# Autodesk Inventor assembly: XL,XC-330
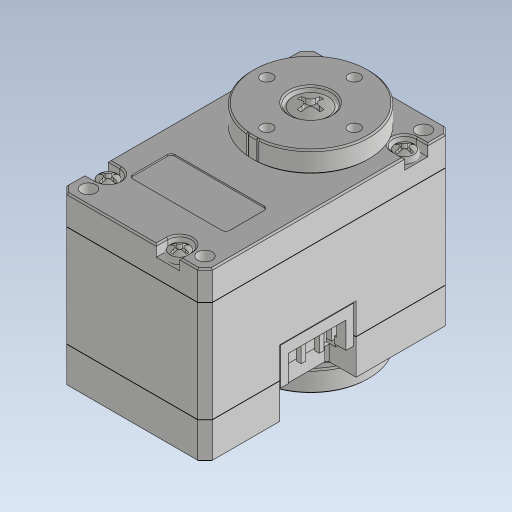
[picture p0: Inventor's stored thumbnail of the model, 512x512]
Saved by Autodesk Inventor 2023 (Build 270158000, 158)
## iProperties
Created: 2020-07-27
Part Number: XL,XC-330
Document SubType Name: Assembly
Designer: michi
Sending System: CREO PARAMETRIC BY PTC INC, 2019224
Preprocessor: CREO PARAMETRIC BY PTC INC, 2019224
Title: DC15_A01_DUMMY_ASSY_IDLE_ASM
Author: yunever
Revision Number: 9LAST_VERSION
## Documents named in this file (11)
- C:\Users\michi\OneDrive - Kyoto University\lab\6_SHINOBI\FUHGA4\Design_Mechanism\Dynamixel\X330\XL,XC-330.iam
- C:\Users\michi\OneDrive - Kyoto University\lab\6_SHINOBI\FUHGA4\Design_Mechanism\Dynamixel\X330\DC15_A01_CASE_M_DUMMY.ipt
- C:\Users\michi\OneDrive - Kyoto University\lab\6_SHINOBI\FUHGA4\Design_Mechanism\Dynamixel\X330\DC15_A01_CASE_F_DUMMY.ipt
- C:\Users\michi\OneDrive - Kyoto University\lab\6_SHINOBI\FUHGA4\Design_Mechanism\Dynamixel\X330\DC15_A01_CASE_B_DUMMY.ipt
- C:\Users\michi\OneDrive - Kyoto University\lab\6_SHINOBI\FUHGA4\Design_Mechanism\Dynamixel\X330\DC15_A01_HORN_DUMMY.ipt
- C:\Users\michi\OneDrive - Kyoto University\lab\6_SHINOBI\FUHGA4\Design_Mechanism\Dynamixel\X330\DC15_A01_LED_CAP2_DUMMY.ipt
- C:\Users\michi\OneDrive - Kyoto University\lab\6_SHINOBI\FUHGA4\Design_Mechanism\Dynamixel\X330\PHS_1_7X20_5_DC10.ipt
- C:\Users\michi\OneDrive - Kyoto University\lab\6_SHINOBI\FUHGA4\Design_Mechanism\Dynamixel\X330\BTS2_M2_6X8.ipt
- C:\Users\michi\OneDrive - Kyoto University\lab\6_SHINOBI\FUHGA4\Design_Mechanism\Dynamixel\X330\DC15_A01_HORN_IDLE2_DUMMY.ipt
- C:\Users\michi\OneDrive - Kyoto University\lab\6_SHINOBI\FUHGA4\Design_Mechanism\Dynamixel\X330\DC15_A01_IDLE_CAP_DUMMY.ipt
- C:\Users\michi\OneDrive - Kyoto University\lab\6_SHINOBI\FUHGA4\Design_Mechanism\Dynamixel\X330\B3B-EH.ipt
## Components (15 placed, 15 different names)
1. 0 — 挿入:2
2. 1
3. 2
4. 3 — 挿入:2
5. 4
6. 5
7. 6
8. 7
9. 8
10. 9
11. 10 — 挿入:1
12. 11 — 挿入:1
13. 12
14. 13
15. 14
## Relationships (2: Insert 2)
- 挿入:1 [Insert]: 10 ↔ 11
- 挿入:2 [Insert]: 0 ↔ 3
